# Autodesk Inventor assembly: s-assy-link1
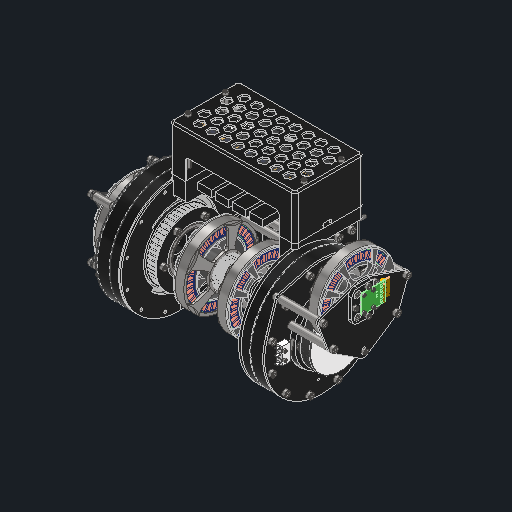
[picture p0: Inventor's stored thumbnail of the model, 512x512]
Saved by Autodesk Inventor 2022 (Build 260153000, 153)
## iProperties
Created: 2021-07-30
Part Number: s-assy-link1
Document SubType Name: Assembly
Designer: yuta0
Mass: 3538.26 g
Surface Area: 7812.66 cm^2
Volume: 1180.98 cm^3
Density: 2.99603 g/cm^3
Author: yuta0
## Documents named in this file (18)
- C:\Users\yuta0\Documents\GitHub\catchrobo_hardware\assy-robot\s-assy-link1.iam
- C:\Users\yuta0\Documents\GitHub\catchrobo_hardware\assy-robot\steel_plate3.ipt
- C:\Users\yuta0\Documents\GitHub\catchrobo_hardware\assy-robot\s-assy-motor-wrist3.iam
- C:\Users\yuta0\Documents\GitHub\catchrobo_hardware\assy-robot\s-assy-unit-j2.iam
- C:\Users\yuta0\Documents\GitHub\catchrobo_hardware\assy-robot\s-assy-unit-j3.iam
- C:\Users\yuta0\Documents\GitHub\catchrobo_hardware\assy-robot\CB4-6.ipt
- C:\Users\yuta0\Documents\GitHub\catchrobo_hardware\assy-robot\SFHRW8-75_7-M4-N4_s.ipt
- C:\Users\yuta0\Documents\GitHub\catchrobo_hardware\assy-robot\SFHRW8-137-M4-N4_s.ipt
- C:\Users\yuta0\Documents\GitHub\catchrobo_hardware\assy-robot\ODrive3.4.ipt
- C:\Users\yuta0\Documents\GitHub\catchrobo_hardware\assy-robot\base44.ipt
- C:\Users\yuta0\Documents\GitHub\catchrobo_hardware\assy-robot\base45.ipt
- C:\Users\yuta0\Documents\GitHub\catchrobo_hardware\assy-robot\base9_2.ipt
- C:\Users\yuta0\Documents\GitHub\catchrobo_hardware\assy-robot\U3H-FC03BBK.ipt
- C:\Users\yuta0\Documents\GitHub\catchrobo_hardware\assy-robot\50wr5j cement resistor.ipt
- C:\Users\yuta0\Documents\GitHub\catchrobo_hardware\assy-robot\hexagonal_spacer_M3_15mm.ipt
- C:\Users\yuta0\Documents\GitHub\catchrobo_hardware\assy-robot\CB4-20.ipt
- C:\Users\yuta0\Documents\GitHub\catchrobo_hardware\assy-robot\CB3-5.ipt
- C:\Users\yuta0\Documents\GitHub\catchrobo_hardware\assy-robot\CB4-50.ipt
## Components (56 placed, 17 different names)
1. steel_plate3:1 — メイト:7, メイト:8, メイト:9, メイト:10, メイト:11, メイト:12, メイト:13, メイト:14, メイト:15, メイト:16, メイト:17, メイト:18, メイト:38, メイト:39, メイト:40, メイト:41, メイト:42, メイト:55, メイト:56, メイト:57, メイト:58, メイト:59, メイト:60, メイト:71, メイト:77, メイト:78, メイト:83, メイト:84, メイト:85, メイト:86
2. s-assy-motor-wrist3:1 [sub-assembly] — メイト:13, メイト:15, メイト:17, メイト:54
3. s-assy-motor-wrist3:2 [sub-assembly] — メイト:14, メイト:16, メイト:18, メイト:34, メイト:35, メイト:36, メイト:37, メイト:45, メイト:46, メイト:47, メイト:48
4. s-assy-unit-j2:1 [sub-assembly] — メイト:7, メイト:8, メイト:9, メイト:69
5. s-assy-unit-j3:1 [sub-assembly] — メイト:10, メイト:11, メイト:12, メイト:79
6. base9_2:1 — メイト:38, メイト:39, メイト:40
7. base44:2 — メイト:69, メイト:70, メイト:71, メイト:73, メイト:76, メイト:81, メイト:82, メイト:90, メイト:91, メイト:92
8. base45:1 — メイト:74, メイト:75, メイト:76, メイト:87, メイト:88, メイト:89, メイト:92, メイト:93, メイト:94, メイト:95, メイト:96, メイト:97
9. U3H-FC03BBK:1 — メイト:77
10. SFHRW8-137-M4-N4_s:3 — メイト:78, メイト:79
11. 50wr5j cement resistor:2 — メイト:89, メイト:93, メイト:94
12. 50wr5j cement resistor:4 — メイト:95, メイト:96, メイト:97
13. CB4-50:1 — メイト:55, メイト:56
14. CB4-50:2
15. CB4-50:3
16. CB4-50:4
17. CB4-50:5
18. CB4-50:6
19. CB4-6:5 — メイト:41, メイト:42
20. SFHRW8-137-M4-N4_s:1 — メイト:57, メイト:58
21. CB4-6:11 — メイト:59, メイト:60
22. CB4-6:9 — メイト:45, メイト:46
23. CB4-6:10 — メイト:47, メイト:48, メイト:53
24. SFHRW8-75_7-M4-N4_s:1 — メイト:53, メイト:54
25. CB4-6:1 — メイト:34, メイト:35
26. CB4-6:2 — メイト:36, メイト:37
27. CB4-6:12
28. SFHRW8-137-M4-N4_s:2
29. CB4-6:13
30. CB4-6:14
31. CB4-6:15
32. SFHRW8-75_7-M4-N4_s:2
33. CB4-6:16
34. CB4-6:17
35. ODrive3.4:1 — メイト:70, メイト:73
36. ODrive3.4:2 — メイト:74, メイト:75
37. CB4-20:2 — メイト:85, メイト:86, メイト:90
38. CB4-20:1 — メイト:83, メイト:84
39. CB4-20:3
40. CB4-20:4
41. CB3-5:1 — メイト:87, メイト:88
42. CB3-5:2
43. CB3-5:3
44. CB3-5:4
45. hexagonal_spacer_M3_15mm:1 — メイト:81, メイト:82
46. hexagonal_spacer_M3_15mm:2
47. hexagonal_spacer_M3_15mm:3
48. hexagonal_spacer_M3_15mm:4
49. hexagonal_spacer_M3_15mm:5
50. hexagonal_spacer_M3_15mm:6
51. hexagonal_spacer_M3_15mm:7 — メイト:91
52. hexagonal_spacer_M3_15mm:8
53. hexagonal_spacer_M3_15mm:9
54. hexagonal_spacer_M3_15mm:10
55. hexagonal_spacer_M3_15mm:11
56. hexagonal_spacer_M3_15mm:12
## Component patterns: (6 elements, first: CB4-50:1), (2 elements, first: CB4-6:5 + SFHRW8-137-M4-N4_s:1 + CB4-6:11 + CB4-6:9 + CB4-6:10 + SFHRW8-75_7-M4-N4_s:1 + CB4-6:1 + CB4-6:2), (2 elements, first: ODrive3.4:1), (3 elements), (2 elements, first: CB4-20:2 + CB4-20:1), (4 elements, first: CB3-5:1), (4 elements, first: hexagonal_spacer_M3_15mm:1), コンポーネント パターン 7:2 (4 elements), コンポーネント パターン 7:3 (4 elements)
## Relationships (60: Mate 60)
- メイト:7 [Mate]: steel_plate3:1 ↔ s-assy-unit-j2:1
- メイト:8 [Mate]: steel_plate3:1 ↔ s-assy-unit-j2:1
- メイト:9 [Mate]: steel_plate3:1 ↔ s-assy-unit-j2:1
- メイト:10 [Mate]: steel_plate3:1 ↔ s-assy-unit-j3:1
- メイト:11 [Mate]: steel_plate3:1 ↔ s-assy-unit-j3:1
- メイト:12 [Mate]: steel_plate3:1 ↔ s-assy-unit-j3:1
- メイト:13 [Mate]: steel_plate3:1 ↔ s-assy-motor-wrist3:1
- メイト:14 [Mate]: steel_plate3:1 ↔ s-assy-motor-wrist3:2
- メイト:15 [Mate]: steel_plate3:1 ↔ s-assy-motor-wrist3:1
- メイト:16 [Mate]: steel_plate3:1 ↔ s-assy-motor-wrist3:2
- メイト:17 [Mate]: steel_plate3:1 ↔ s-assy-motor-wrist3:1
- メイト:18 [Mate]: steel_plate3:1 ↔ s-assy-motor-wrist3:2
- メイト:34 [Mate]: s-assy-motor-wrist3:2 ↔ CB4-6:1
- メイト:35 [Mate]: s-assy-motor-wrist3:2 ↔ CB4-6:1
- メイト:36 [Mate]: s-assy-motor-wrist3:2 ↔ CB4-6:2
- メイト:37 [Mate]: s-assy-motor-wrist3:2 ↔ CB4-6:2
- メイト:38 [Mate]: steel_plate3:1 ↔ base9_2:1
- メイト:39 [Mate]: steel_plate3:1 ↔ base9_2:1
- メイト:40 [Mate]: steel_plate3:1 ↔ base9_2:1
- メイト:41 [Mate]: steel_plate3:1 ↔ CB4-6:5
- メイト:42 [Mate]: steel_plate3:1 ↔ CB4-6:5
- メイト:45 [Mate]: s-assy-motor-wrist3:2 ↔ CB4-6:9
- メイト:46 [Mate]: s-assy-motor-wrist3:2 ↔ CB4-6:9
- メイト:47 [Mate]: s-assy-motor-wrist3:2 ↔ CB4-6:10
- メイト:48 [Mate]: s-assy-motor-wrist3:2 ↔ CB4-6:10
- メイト:53 [Mate]: CB4-6:10 ↔ SFHRW8-75_7-M4-N4_s:1
- メイト:54 [Mate]: s-assy-motor-wrist3:1 ↔ SFHRW8-75_7-M4-N4_s:1
- メイト:55 [Mate]: steel_plate3:1 ↔ CB4-50:1
- メイト:56 [Mate]: steel_plate3:1 ↔ CB4-50:1
- メイト:57 [Mate]: steel_plate3:1 ↔ SFHRW8-137-M4-N4_s:1
- メイト:58 [Mate]: steel_plate3:1 ↔ SFHRW8-137-M4-N4_s:1
- メイト:59 [Mate]: steel_plate3:1 ↔ CB4-6:11
- メイト:60 [Mate]: steel_plate3:1 ↔ CB4-6:11
- メイト:69 [Mate]: s-assy-unit-j2:1 ↔ base44:2
- メイト:70 [Mate]: base44:2 ↔ ODrive3.4:1
- メイト:71 [Mate]: steel_plate3:1 ↔ base44:2
- メイト:73 [Mate] (15 mm): base44:2 ↔ ODrive3.4:1
- メイト:74 [Mate]: base45:1 ↔ ODrive3.4:2
- メイト:75 [Mate]: base45:1 ↔ ODrive3.4:2
- メイト:76 [Mate]: base44:2 ↔ base45:1
- メイト:77 [Mate]: steel_plate3:1 ↔ U3H-FC03BBK:1
- メイト:78 [Mate]: steel_plate3:1 ↔ SFHRW8-137-M4-N4_s:3
- メイト:79 [Mate]: s-assy-unit-j3:1 ↔ SFHRW8-137-M4-N4_s:3
- メイト:81 [Mate]: base44:2 ↔ hexagonal_spacer_M3_15mm:1
- メイト:82 [Mate]: base44:2 ↔ hexagonal_spacer_M3_15mm:1
- メイト:83 [Mate]: steel_plate3:1 ↔ CB4-20:1
- メイト:84 [Mate]: steel_plate3:1 ↔ CB4-20:1
- メイト:85 [Mate]: steel_plate3:1 ↔ CB4-20:2
- メイト:86 [Mate]: steel_plate3:1 ↔ CB4-20:2
- メイト:87 [Mate]: base45:1 ↔ CB3-5:1
- メイト:88 [Mate]: base45:1 ↔ CB3-5:1
- メイト:89 [Mate]: base45:1 ↔ 50wr5j cement resistor:2
- メイト:90 [Mate]: base44:2 ↔ CB4-20:2
- メイト:91 [Mate]: base44:2 ↔ hexagonal_spacer_M3_15mm:7
- メイト:92 [Mate]: base44:2 ↔ base45:1
- メイト:93 [Mate]: base45:1 ↔ 50wr5j cement resistor:2
- メイト:94 [Mate]: base45:1 ↔ 50wr5j cement resistor:2
- メイト:95 [Mate]: base45:1 ↔ 50wr5j cement resistor:4
- メイト:96 [Mate]: base45:1 ↔ 50wr5j cement resistor:4
- メイト:97 [Mate]: base45:1 ↔ 50wr5j cement resistor:4
